# Autodesk Inventor assembly: Piano
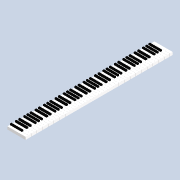
[picture p0: Inventor's stored thumbnail of the model, 180x180]
Saved by Autodesk Inventor 2021 (Build 250183000, 183)
## iProperties
Created: 2021-03-17
Part Number: Piano
Document SubType Name: Assembly
Designer: Tom
Author: Tom
## Documents named in this file (6)
- C:\Users\Tom\Documents\Inventor\Piano\Piano.iam
- C:\Users\Tom\Documents\Inventor\Piano\Octave.iam
- C:\Users\Tom\Documents\Inventor\Piano\Key--Highest.ipt
- C:\Users\Tom\Documents\Inventor\Piano\Key--B.ipt
- C:\Users\Tom\Documents\Inventor\Piano\Key--Lowest.ipt
- C:\Users\Tom\Documents\Inventor\Piano\Key--Black.ipt
## Components (11 placed, 5 different names)
1. Key--Highest:1 — Mate:1, Flush:1, Flush:2
2. Key--B:1 — Mate:2, Flush:3, Flush:4, Mate:3, Flush:5, Flush:6, Flush:7, Mate:4, Flush:8
3. Key--Lowest:1 — Mate:3, Flush:5, Flush:6
4. Key--Black:1 — Flush:7, Mate:4, Flush:8
5. Octave:1 [sub-assembly] — Mate:2, Flush:3, Flush:4
6. Octave:2 [sub-assembly]
7. Octave:3 [sub-assembly]
8. Octave:4 [sub-assembly]
9. Octave:5 [sub-assembly]
10. Octave:6 [sub-assembly]
11. Octave:7 [sub-assembly] — Mate:1, Flush:1, Flush:2
## Component patterns: (7 elements, first: Octave:1)
## Relationships (12: Flush 8, Mate 4)
- Mate:1 (0.7937 mm): Key--Highest:1 ↔ Octave:7
- Flush:1: Key--Highest:1 ↔ Octave:7
- Flush:2: Key--Highest:1 ↔ Octave:7
- Mate:2 (0.7937 mm): Key--B:1 ↔ Octave:1
- Flush:3: Key--B:1 ↔ Octave:1
- Flush:4: Key--B:1 ↔ Octave:1
- Mate:3 (0.7937 mm): Key--B:1 ↔ Key--Lowest:1
- Flush:5: Key--B:1 ↔ Key--Lowest:1
- Flush:6: Key--B:1 ↔ Key--Lowest:1
- Flush:7: Key--B:1 ↔ Key--Black:1
- Mate:4 (0.7937 mm): Key--B:1 ↔ Key--Black:1
- Flush:8: Key--B:1 ↔ Key--Black:1
